# Autodesk Inventor assembly: 134
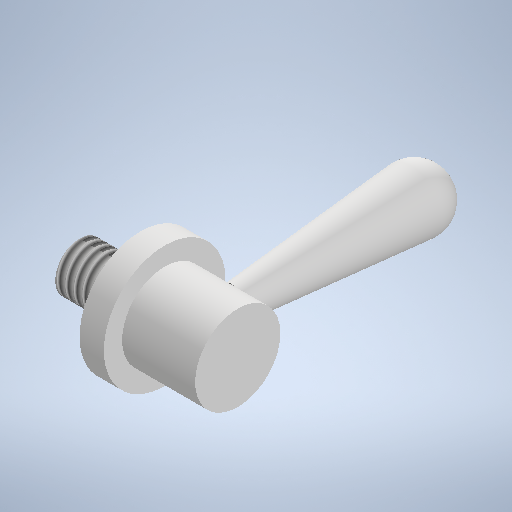
[picture p0: Inventor's stored thumbnail of the model, 512x512]
Saved by Autodesk Inventor 2025.1 (Build 291241000, 241)
## iProperties
Created: 2024-08-05
Part Number: 134
Document SubType Name: Assembly
Designer: ffogue
Author: ffogue
## Documents named in this file (3)
- C:\Projkete - Übungen\Freedom\134.iam
- C:\Projkete - Übungen\Freedom\134 handle.ipt
- C:\Projkete - Übungen\Freedom\134.ipt
## Components (2 placed, 2 different names)
1. 134 handle:1 — Mate:1, Insert:1
2. 134:1 — Mate:1, Insert:1
## Relationships (2: Mate 1, Insert 1)
- Mate:1: 134 handle:1 ↔ 134:1
- Insert:1: 134 handle:1 ↔ 134:1
